# Autodesk Inventor assembly: Left Side Tower Assembly_MIR
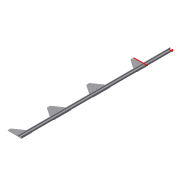
[picture p0: Inventor's stored thumbnail of the model, 180x180]
Saved by Autodesk Inventor 2015 (Build 190159000, 159)
## iProperties
Created: 2015-01-24
Part Number: Left Side Tower Assembly_MIR
Document SubType Name: Assembly
Designer: Peter
Author: Peter
## Documents named in this file (4)
- C:\Users\Tanner\Documents\GitHub\FIRST-Team-1719-CAD-Team\2015 Robot CAD\Lifter Super Structure\Tower\Side-Towers Assemblies\Left Side Tower Assembly_MIR.iam
- C:\Users\Tanner\Documents\GitHub\FIRST-Team-1719-CAD-Team\2015 Robot CAD\Lifter Super Structure\Tower\Side-Towers Assemblies\Vertical-Unistrut-Tower-75_MIR.ipt
- C:\Users\Tanner\Documents\GitHub\FIRST-Team-1719-CAD-Team\2015 Robot CAD\Lifter Super Structure\Tower\Side-Towers Assemblies\Center-Tower-Brace_MIR.ipt
- C:\Users\Tanner\Documents\GitHub\FIRST-Team-1719-CAD-Team\2015 Robot CAD\Lifter Super Structure\Tower\Side-Towers Assemblies\Corner-Tower-Brace_MIR.ipt
## Components (5 placed, 3 different names)
1. Vertical-Unistrut-Tower-75_MIR:1 — Flush:9, Mate:8, Flush:8, Mate:9, Flush:1, Flush:10, Mate:7, Flush:7, Flush:11, Mate:6, Flush:6
2. Center-Tower-Brace_MIR:1 — Flush:9, Mate:8, Mate:5
3. Corner-Tower-Brace_MIR:1 — Flush:8, Mate:9, Mate:5, Flush:1
4. Center-Tower-Brace_MIR:2 — Flush:10, Mate:7, Flush:7
5. Corner-Tower-Brace_MIR:2 — Flush:11, Mate:6, Flush:6
## Relationships (12: Flush 7, Mate 5)
- Flush:9: Vertical-Unistrut-Tower-75_MIR:1 ↔ Center-Tower-Brace_MIR:1
- Mate:8: Vertical-Unistrut-Tower-75_MIR:1 ↔ Center-Tower-Brace_MIR:1
- Flush:8: Vertical-Unistrut-Tower-75_MIR:1 ↔ Corner-Tower-Brace_MIR:1
- Mate:9: Vertical-Unistrut-Tower-75_MIR:1 ↔ Corner-Tower-Brace_MIR:1
- Mate:5 (269.0495 mm): Center-Tower-Brace_MIR:1 ↔ Corner-Tower-Brace_MIR:1
- Flush:1: Vertical-Unistrut-Tower-75_MIR:1 ↔ Corner-Tower-Brace_MIR:1
- Flush:10: Vertical-Unistrut-Tower-75_MIR:1 ↔ Center-Tower-Brace_MIR:2
- Mate:7: Vertical-Unistrut-Tower-75_MIR:1 ↔ Center-Tower-Brace_MIR:2
- Flush:7 (-774.7 mm): Vertical-Unistrut-Tower-75_MIR:1 ↔ Center-Tower-Brace_MIR:2
- Flush:11: Vertical-Unistrut-Tower-75_MIR:1 ↔ Corner-Tower-Brace_MIR:2
- Mate:6: Vertical-Unistrut-Tower-75_MIR:1 ↔ Corner-Tower-Brace_MIR:2
- Flush:6 (-311.15 mm): Vertical-Unistrut-Tower-75_MIR:1 ↔ Corner-Tower-Brace_MIR:2
